# Autodesk Inventor assembly: FullView
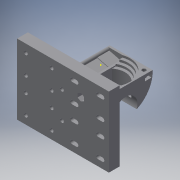
[picture p0: Inventor's stored thumbnail of the model, 180x180]
Saved by Autodesk Inventor 2019 (Build 230136000, 136)
## iProperties
Created: 2018-06-29
Part Number: FullView
Material: Ogólny
Document SubType Name: Assembly
Designer: Kamil
Author: Kamil
## Documents named in this file (4)
- D:\Git\3DPrinting\E3DExtruderHolder\FullView.iam
- D:\Git\3DPrinting\E3DExtruderHolder\ExtruderHolder.ipt
- D:\Git\3DPrinting\E3DExtruderHolder\ExtruderCooler.ipt
- D:\Git\3DPrinting\E3DExtruderHolder\ExtruderClamp.ipt
## Components (3 placed, 3 different names)
1. ExtruderCooler:1
2. ExtruderClamp:1 — Walcowe:1
3. ExtruderHolder:1 — Walcowe:1
## Relationships (1: CylindricalJoint 1)
- Walcowe:1 [CylindricalJoint]: ExtruderClamp:1 ↔ ExtruderHolder:1
